# Autodesk Inventor assembly: bubinek_sestava
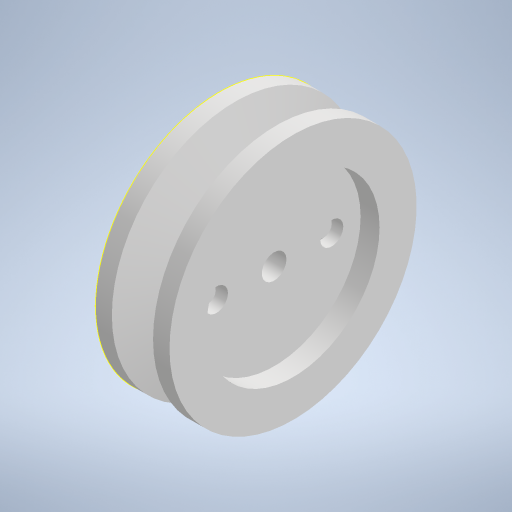
[picture p0: Inventor's stored thumbnail of the model, 512x512]
Saved by Autodesk Inventor 2023.1 (Build 271208000, 208)
## iProperties
Created: 2023-01-10
Part Number: bubinek_sestava
Document SubType Name: Assembly
Designer: zavrel
Author: zavrel
## Documents named in this file (3)
- C:\Users\zavrel\Documents\_OWNCLOUD_ACTUAL_WORK\GACR_Tensegrity\35_pohon_pro_Miletin\sestava_pohonu_SERVO\bubinek_sestava.iam
- C:\Users\zavrel\Documents\_OWNCLOUD_ACTUAL_WORK\GACR_Tensegrity\35_pohon_pro_Miletin\sestava_pohonu_SERVO\bubinek_BOTTOM.ipt
- C:\Users\zavrel\Documents\_OWNCLOUD_ACTUAL_WORK\GACR_Tensegrity\35_pohon_pro_Miletin\sestava_pohonu_SERVO\bubinek_TOP.ipt
## Components (2 placed, 2 different names)
1. bubinek_BOTTOM:1 — Rigid:2
2. bubinek_TOP:1 — Rigid:2
## Relationships (1: WeldJoint 1)
- Rigid:2 [WeldJoint]: bubinek_BOTTOM:1 ↔ bubinek_TOP:1
